# Autodesk Inventor assembly: Trippeldekker_Assembly_V2
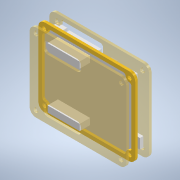
[picture p0: Inventor's stored thumbnail of the model, 180x180]
Saved by Autodesk Inventor 2022 (Build 260153000, 153)
## iProperties
Created: 2021-08-29
Part Number: Trippeldekker_Assembly_V2
Document SubType Name: Assembly
Designer: Bruker
Author: Bruker
## Documents named in this file (5)
- D:\Inventor\MSP430 Etui\Versjon 2\Mikrokontroller_boks\Trippeldekker_Assembly_V2.iam
- D:\Inventor\MSP430 Etui\Versjon 2\Mikrokontroller_boks\Trippeldekker_Midtre plate.ipt
- D:\Inventor\MSP430 Etui\Versjon 2\Mikrokontroller_boks\Trippeldekker_Nedre plate.ipt
- D:\Inventor\MSP430 Etui\Versjon 2\Mikrokontroller_boks\Trippeldekker_Øvre plate.ipt
- D:\Inventor\MSP430 Etui\Versjon 2\lunchpad.0006.ipt
## Components (4 placed, 4 different names)
1. Trippeldekker_Midtre plate:1 — Rotational:1, Rotational:2, Rotational:3
2. Trippeldekker_Nedre plate:1 — Rotational:1
3. Trippeldekker_Øvre plate:1 — Rotational:2
4. lunchpad.0006:1 — Rotational:3
## Relationships (3: RevoluteJoint 3)
- Rotational:1 [RevoluteJoint] (7 mm): Trippeldekker_Midtre plate:1 ↔ Trippeldekker_Nedre plate:1
- Rotational:2 [RevoluteJoint] (8 mm): Trippeldekker_Midtre plate:1 ↔ Trippeldekker_Øvre plate:1
- Rotational:3 [RevoluteJoint] (2 mm): Trippeldekker_Midtre plate:1 ↔ lunchpad.0006:1
